# Autodesk Inventor assembly: Project_1M
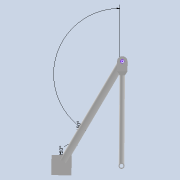
[picture p0: Inventor's stored thumbnail of the model, 180x180]
Saved by Autodesk Inventor 2021 (Build 250183000, 183)
## iProperties
Created: 2022-04-30
Part Number: Project_1M
Document SubType Name: Assembly
Designer: jgarn
Sending System: Autodesk Inventor 2022
Preprocessor: ST-DEVELOPER v18.1
Title: C:\Users\Jhon Brando\Documents\Servomecanismo\Project_1M.stp
Author: Jhon Brando
## Documents named in this file (4)
- C:\Users\jgarn\Documents\Proyectos Servos\Proyecto Academico\Modelo CAD\Project_1M.iam
- C:\Users\jgarn\Documents\Proyectos Servos\Proyecto Academico\Modelo CAD\Link_1M.ipt
- C:\Users\jgarn\Documents\Proyectos Servos\Proyecto Academico\Modelo CAD\Link_2M.ipt
- C:\Users\jgarn\Documents\Proyectos Servos\Proyecto Academico\Modelo CAD\BaseM.ipt
## Components (3 placed, 3 different names)
1. Link_1:1 — Rotational:1, Rotational:2
2. Link_2:1 — Rotational:2
3. Base:2 — Rotational:1
## Relationships (2: RevoluteJoint 2)
- Rotational:1 [RevoluteJoint]: Link_1:1 ↔ Base:2
- Rotational:2 [RevoluteJoint]: Link_1:1 ↔ Link_2:1
